# Autodesk Inventor assembly: base_assembly
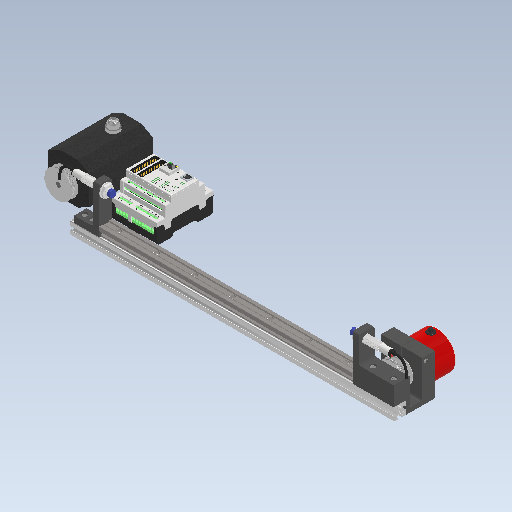
[picture p0: Inventor's stored thumbnail of the model, 512x512]
Saved by Autodesk Inventor 2021 (Build 250183000, 183)
## iProperties
Created: 2022-07-01
Part Number: base_assembly
Document SubType Name: Assembly
Designer: lenna
Author: lenna
## Documents named in this file (16)
- C:\Users\lenna\Desktop\Lennart\Uni\Master\2. Semester\SDM\CAD_neu\base_assembly.iam
- C:\Users\lenna\Desktop\Lennart\Uni\Master\2. Semester\SDM\CAD_neu\item_profile.ipt
- C:\Users\lenna\Desktop\Lennart\Uni\Master\2. Semester\SDM\CAD_neu\rail.ipt
- C:\Users\lenna\Desktop\Lennart\Uni\Master\2. Semester\SDM\CAD_neu\pulley_positioner.ipt
- C:\Users\lenna\Desktop\Lennart\Uni\Master\2. Semester\SDM\CAD_neu\inductive_sensor_adapter.ipt
- C:\Users\lenna\Desktop\Lennart\Uni\Master\2. Semester\SDM\CAD_neu\inductive_sensor.ipt
- C:\Users\lenna\Desktop\Lennart\Uni\Master\2. Semester\SDM\CAD_neu\opkon_encoder.ipt
- C:\Users\lenna\Desktop\Lennart\Uni\Master\2. Semester\SDM\CAD_neu\gt2_60.ipt
- C:\Users\lenna\Desktop\Lennart\Uni\Master\2. Semester\SDM\CAD_neu\controllino_maxi_automation.ipt
- C:\Users\lenna\Desktop\Lennart\Uni\Master\2. Semester\SDM\CAD_neu\dunkermotor.ipt
- C:\Users\lenna\Desktop\Lennart\Uni\Master\2. Semester\SDM\CAD_neu\M3_threaded_rod_70.ipt
- C:\Users\lenna\Desktop\Lennart\Uni\Master\2. Semester\SDM\CAD_neu\M4_groove_stone.ipt
- C:\Users\lenna\Documents\Inventor\Content Center Files\R2021\en-US\ISO 4762(1)\DIN EN ISO 4762 - M4 x 30.ipt
- C:\Users\lenna\Documents\Inventor\Content Center Files\R2021\en-US\ISO 4762(1)\DIN EN ISO 4762 - M4 x 10.ipt
- C:\Users\lenna\Documents\Inventor\Content Center Files\R2021\en-US\ISO 4762(1)\DIN EN ISO 4762 - M4 x 16.ipt
- C:\Users\lenna\Documents\Inventor\Content Center Files\R2021\en-US\DIN EN ISO 4035\DIN EN ISO 4035 - M3.ipt
## Components (37 placed, 15 different names)
1. item_profile:1 — Mate:1, Mate:2, Flush:1, Mate:3, Mate:4, Mate:5, Flush:2, Flush:3, Mate:6, Mate:7, Flush:4
2. item_profile:2 — Mate:5, Flush:2, Flush:3, Mate:9, Flush:5
3. rail:1 — Mate:3, Mate:4, Mate:8, Mate:10, Insert:12
4. pulley_positioner:1 — Mate:6, Mate:7, Flush:4, Mate:8, Insert:1, Insert:3, Insert:6, Insert:8, Insert:13, Insert:14
5. inductive_sensor_adapter:1 — Mate:9, Flush:5, Mate:10, Insert:4, Insert:10
6. inductive_sensor:1 — Insert:3, Angle:2
7. inductive_sensor:2 — Insert:4, Angle:3
8. opkon_encoder:1 — Insert:1, Angle:1, Insert:2
9. gt2_60:1 — Insert:2, Flush:6
10. gt2_60:2 — Insert:5, Flush:6
11. dunkermotor:1 — Mate:11, Insert:5, Mate:13
12. controllino_maxi_automation:1 — Mate:12, Mate:13
13. M3_threaded_rod_70:1 — Insert:6
14. DIN EN ISO 4035 M3:1 — Insert:13
15. DIN EN ISO 4035 M3:2 — Insert:14
16. DIN EN ISO 4762 M4 x 30:1 — Insert:7, Insert:8
17. M4_groove_stone:1 — Insert:7
18. DIN EN ISO 4762 M4 x 30:2
19. M4_groove_stone:2
20. DIN EN ISO 4762 M4 x 10:1 — Insert:10
21. M4_groove_stone:3
22. DIN EN ISO 4762 M4 x 10:2
23. M4_groove_stone:4
24. DIN EN ISO 4762 M4 x 16:1 — Insert:12
25. M4_groove_stone:5
26. DIN EN ISO 4762 M4 x 16:2
27. M4_groove_stone:6
28. DIN EN ISO 4762 M4 x 16:3
29. M4_groove_stone:7
30. DIN EN ISO 4762 M4 x 16:4
31. M4_groove_stone:8
32. DIN EN ISO 4762 M4 x 16:5
33. M4_groove_stone:9
34. DIN EN ISO 4762 M4 x 16:6
35. M4_groove_stone:10
36. DIN EN ISO 4762 M4 x 16:7
37. M4_groove_stone:11
## Component patterns: (2 elements, first: DIN EN ISO 4762 M4 x 30:1 + M4_groove_stone:1), (2 elements, first: DIN EN ISO 4762 M4 x 10:1 + M4_groove_stone:3), (7 elements, first: DIN EN ISO 4762 M4 x 16:1 + M4_groove_stone:5)
## Relationships (36: Insert 14, Mate 13, Flush 6, Angle 3)
- Mate:1: item_profile:1
- Mate:2: item_profile:1
- Flush:1: item_profile:1
- Mate:3: item_profile:1 ↔ rail:1
- Mate:4: item_profile:1 ↔ rail:1
- Mate:5: item_profile:1 ↔ item_profile:2
- Flush:2: item_profile:1 ↔ item_profile:2
- Flush:3: item_profile:1 ↔ item_profile:2
- Mate:6: item_profile:1 ↔ pulley_positioner:1
- Mate:7: item_profile:1 ↔ pulley_positioner:1
- Flush:4: item_profile:1 ↔ pulley_positioner:1
- Mate:8: rail:1 ↔ pulley_positioner:1
- Insert:1: pulley_positioner:1 ↔ opkon_encoder:1
- Angle:1 (0 deg): opkon_encoder:1
- Insert:2 (1 mm): opkon_encoder:1 ↔ gt2_60:1
- Insert:3: pulley_positioner:1 ↔ inductive_sensor:1
- Angle:2 (180 deg): inductive_sensor:1
- Mate:9: item_profile:2 ↔ inductive_sensor_adapter:1
- Flush:5: item_profile:2 ↔ inductive_sensor_adapter:1
- Mate:10: rail:1 ↔ inductive_sensor_adapter:1
- Insert:4: inductive_sensor_adapter:1 ↔ inductive_sensor:2
- Angle:3 (0 deg): inductive_sensor:2
- Mate:11: dunkermotor:1
- Mate:12: controllino_maxi_automation:1
- Insert:5: gt2_60:2 ↔ dunkermotor:1
- Flush:6: gt2_60:1 ↔ gt2_60:2
- Mate:13 (25 mm): dunkermotor:1 ↔ controllino_maxi_automation:1
- Insert:6 (-2.5 mm): pulley_positioner:1 ↔ M3_threaded_rod_70:1
- Insert:7 (1 mm): DIN EN ISO 4762 M4 x 30:1 ↔ M4_groove_stone:1
- Insert:8: pulley_positioner:1 ↔ DIN EN ISO 4762 M4 x 30:1
- [Insert] (1 mm): DIN EN ISO 4762 M4 x 10:1 ↔ M4_groove_stone:3
- Insert:10: inductive_sensor_adapter:1 ↔ DIN EN ISO 4762 M4 x 10:1
- [Insert] (1 mm): DIN EN ISO 4762 M4 x 16:1 ↔ M4_groove_stone:5
- Insert:12: rail:1 ↔ DIN EN ISO 4762 M4 x 16:1
- Insert:13: pulley_positioner:1 ↔ DIN EN ISO 4035 M3:1
- Insert:14: pulley_positioner:1 ↔ DIN EN ISO 4035 M3:2
## Named parameters: d37_d31 = 1 mm, d43_d31 = 1 mm
